# Autodesk Inventor assembly: Simple_Body
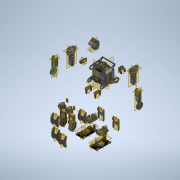
[picture p0: Inventor's stored thumbnail of the model, 180x180]
Saved by Autodesk Inventor 2022.5 (Build 265521000, 521)
## iProperties
Created: 2023-09-11
Part Number: Simple_Body
Document SubType Name: Assembly
Designer: Masato Kubotera
Author: Masato Kubotera
## Documents named in this file (20)
- C:\Users\Masato\Documents\Inventor\SUSTAINA-OP\SimplifiedModelFiles\Simple_Body.iam
- C:\Users\Masato\Documents\Inventor\SUSTAINA-OP\SimplifiedModelFiles\Simple_Ankle.ipt
- C:\Users\Masato\Documents\Inventor\SUSTAINA-OP\SimplifiedModelFiles\Simple_BackLowerLink.ipt
- C:\Users\Masato\Documents\Inventor\SUSTAINA-OP\SimplifiedModelFiles\Simple_BackUpperLink.ipt
- C:\Users\Masato\Documents\Inventor\SUSTAINA-OP\SimplifiedModelFiles\Simple_Foot.ipt
- C:\Users\Masato\Documents\Inventor\SUSTAINA-OP\SimplifiedModelFiles\Simple_ForeArm.ipt
- C:\Users\Masato\Documents\Inventor\SUSTAINA-OP\SimplifiedModelFiles\Simple_Head.ipt
- C:\Users\Masato\Documents\Inventor\SUSTAINA-OP\SimplifiedModelFiles\Simple_Knee.ipt
- C:\Users\Masato\Documents\Inventor\SUSTAINA-OP\SimplifiedModelFiles\Simple_Leg_joint_roll_pitch.ipt
- C:\Users\Masato\Documents\Inventor\SUSTAINA-OP\SimplifiedModelFiles\Simple_Leg_joint_roll_yaw.ipt
- C:\Users\Masato\Documents\Inventor\SUSTAINA-OP\SimplifiedModelFiles\Simple_Shoulder.ipt
- C:\Users\Masato\Documents\Inventor\SUSTAINA-OP\SimplifiedModelFiles\Simple_Trunk.ipt
- C:\Users\Masato\Documents\Inventor\SUSTAINA-OP\SimplifiedModelFiles\Simple_UpperArm.ipt
- C:\Users\Masato\Documents\Inventor\SUSTAINA-OP\SimplifiedModelFiles\Simple_FrontLink.ipt
- C:\Users\Masato\Documents\Inventor\SUSTAINA-OP\SimplifiedModelFiles\Simple_Ankle_MIR.ipt
- C:\Users\Masato\Documents\Inventor\SUSTAINA-OP\SimplifiedModelFiles\Simple_Foot_MIR.ipt
- C:\Users\Masato\Documents\Inventor\SUSTAINA-OP\SimplifiedModelFiles\Simple_Knee_MIR.ipt
- C:\Users\Masato\Documents\Inventor\SUSTAINA-OP\SimplifiedModelFiles\Simple_UpperArm_MIR.ipt
- C:\Users\Masato\Documents\Inventor\SUSTAINA-OP\SimplifiedModelFiles\Simple_Slider_crank_mechanism.ipt
- C:\Users\Masato\Documents\Inventor\SUSTAINA-OP\SimplifiedModelFiles\Simple_Ankle_independent_pitch.ipt
## Components (30 placed, 19 different names)
1. Simple_Head:1
2. Simple_Trunk:1
3. Simple_Shoulder:1
4. Simple_Shoulder:2
5. Simple_UpperArm:1
6. Simple_UpperArm_MIR:1
7. Simple_ForeArm:1
8. Simple_ForeArm:2
9. Simple_Leg_joint_roll_yaw:1
10. Simple_Leg_joint_roll_yaw:2
11. Simple_Leg_joint_roll_pitch:1
12. Simple_Leg_joint_roll_pitch:2
13. Simple_Knee:1
14. Simple_Knee_MIR:1
15. Simple_FrontLink:1
16. Simple_FrontLink:2
17. Simple_FrontLink:3
18. Simple_FrontLink:4
19. Simple_BackUpperLink:1
20. Simple_BackUpperLink:2
21. Simple_BackLowerLink:1
22. Simple_BackLowerLink:2
23. Simple_Ankle:1 — メイト:1
24. Simple_Ankle_MIR:1
25. Simple_Foot:1
26. Simple_Foot_MIR:1
27. Simple_Slider_crank_mechanism:1
28. Simple_Slider_crank_mechanism:2
29. Simple_Ankle_independent_pitch:1 — メイト:1
30. Simple_Ankle_independent_pitch:2
## Relationships (1: Mate 1)
- メイト:1 [Mate]: Simple_Ankle:1 ↔ Simple_Ankle_independent_pitch:1
